# Autodesk Inventor assembly: POLOLU+mocowanie
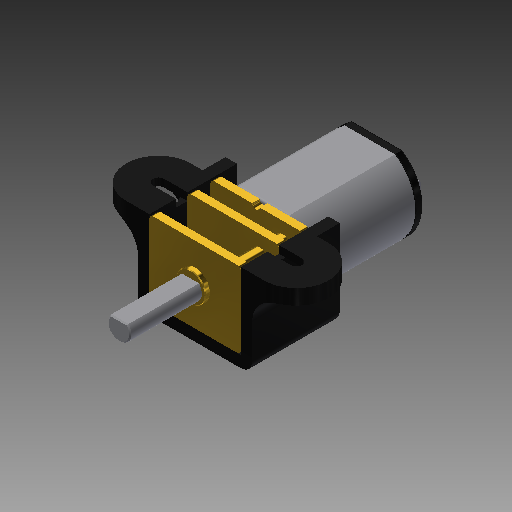
[picture p0: Inventor's stored thumbnail of the model, 512x512]
Saved by Autodesk Inventor 2017 (Build 210142000, 142)
## iProperties
Created: 2016-11-09
Part Number: POLOLU+mocowanie
Document SubType Name: Assembly
Designer: Shichi
Author: Shichi
## Documents named in this file (3)
- C:\Users\Shichi\Desktop\TooStronk\POLOLU+mocowanie.iam
- C:\Users\Shichi\Desktop\TooStronk\Mocowanie_POLOLU.ipt
- C:\Users\Shichi\Desktop\TooStronk\POLOLU.ipt
## Components (2 placed, 2 different names)
1. Mocowanie_POLOLU:1 — Mate:1, Mate:2
2. POLOLU:1 — Mate:1, Mate:2
## Relationships (2: Mate 2)
- Mate:1: Mocowanie_POLOLU:1 ↔ POLOLU:1
- Mate:2: Mocowanie_POLOLU:1 ↔ POLOLU:1
